# Autodesk Inventor assembly: Servo-Bracket Assembly
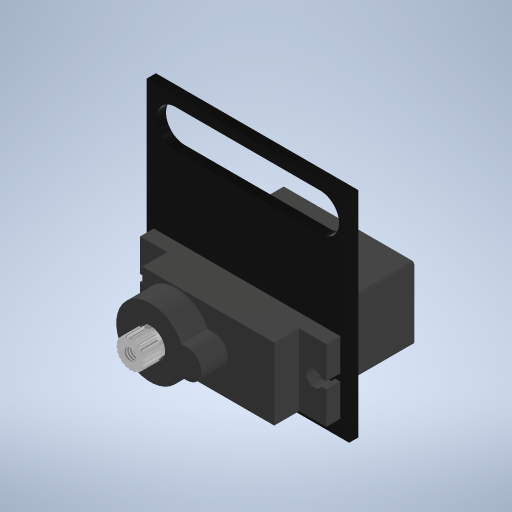
[picture p0: Inventor's stored thumbnail of the model, 512x512]
Saved by Autodesk Inventor 2023 (Build 270158000, 158)
## iProperties
Created: 2022-10-04
Part Number: Servo-Bracket Assembly
Document SubType Name: Assembly
Designer: Raker
Author: Raker
## Documents named in this file (3)
- D:\College Stuff\ATMAE Robotics\Pill Dispenser Robot\Electronics\Servos\OldVersions\Servo-Bracket Assembly.iam
- D:\College Stuff\ATMAE Robotics\Pill Dispenser Robot\Plates and Brackets\Servo_mount_flat.ipt
- D:\College Stuff\ATMAE Robotics\Pill Dispenser Robot\Electronics\Servos\MG90S Servo Motor.ipt
## Components (2 placed, 2 different names)
1. Servo_mount_flat:1 — Mate:1, Mate:2, Mate:3
2. MG90S Servo Motor:1 — Mate:1, Mate:2, Mate:3
## Relationships (3: Mate 3)
- Mate:1: Servo_mount_flat:1 ↔ MG90S Servo Motor:1
- Mate:2: Servo_mount_flat:1 ↔ MG90S Servo Motor:1
- Mate:3: Servo_mount_flat:1 ↔ MG90S Servo Motor:1
